# Autodesk Inventor assembly: Gearbox #2
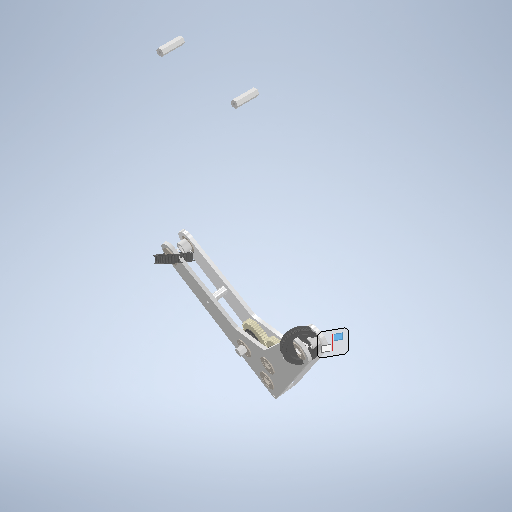
[picture p0: Inventor's stored thumbnail of the model, 512x512]
Saved by Autodesk Inventor 2025.1 (Build 291241020, 241B)
## iProperties
Created: 2024-09-29
Part Number: Gearbox #2
Document SubType Name: Assembly
Designer: xmand
Author: xmand
## Documents named in this file (13)
- C:\Users\xmand\OneDrive\Documents\GitHub\1622-2024-Assignments\Xavier Daza\Gearbox #2.iam
- C:\Users\xmand\OneDrive\Documents\GitHub\1622-2024-Assignments\Xavier Daza\Gearbox #1\Gearbox #2 Top Plate.ipt
- C:\Users\xmand\OneDrive\Documents\GitHub\1622-2024-Assignments\Xavier Daza\Gearbox #1\Gearbox #2 Plate.ipt
- C:\Users\xmand\OneDrive\Documents\GitHub\1622-2024-Assignments\Xavier Daza\Gearbox #1\WCP-0188 (1).ipt
- C:\Users\xmand\Downloads\WCP-0709\WCP-0709\WCP-0709.ipt
- C:\Users\xmand\Downloads\WCP-0783\WCP-0783\WCP-0783.ipt
- C:\Users\xmand\Downloads\WCP-0564\WCP-0564\WCP-0564.ipt
- C:\Users\xmand\Downloads\WCP-0990\WCP-0990\WCP-0990.ipt
- C:\Users\xmand\OneDrive\Documents\GitHub\1622-2024-Assignments\Xavier Daza\WCP-0787-01.ipt
- C:\Users\xmand\OneDrive\Documents\GitHub\1622-2024-Assignments\Xavier Daza\10-32 0.5 1.131 Inch Stand Off.ipt
- C:\Users\xmand\OneDrive\Documents\GitHub\1622-2024-Assignments\Xavier Daza\0.498 Spacer 0.5 Hex.ipt
- C:\Users\xmand\OneDrive\Documents\GitHub\1622-2024-Assignments\Xavier Daza\0.633 Spacer 0.5 Hex.ipt
- C:\Users\xmand\OneDrive\Documents\GitHub\1622-2024-Assignments\Xavier Daza\Hex shaft 0.201 and 0.500.ipt
## Components (32 placed, 12 different names)
1. Gearbox #2 Top Plate:1 — Mate:1, Mate:2, Insert:6, Insert:7, Insert:8, Insert:9, Insert:10, Mate:17, Mate:18, Mate:19
2. Gearbox #2 Plate:1 — Mate:1, Mate:2, Insert:1, Insert:2, Insert:3, Insert:4, Insert:5, Mate:15, Mate:16
3. WCP-0188 (1):1 — Mate:5, Angle:2, Angle:4, Mate:7, Angle:8
4. WCP-0188 (1):2 — Mate:3, Angle:1, Angle:5, Mate:6, Angle:10
5. WCP-0709:1 — Mate:4, Angle:3, Angle:6
6. WCP-0783:1 — Insert:7, Angle:4, Mate:10
7. WCP-0783:2 — Insert:4, Mate:4, Angle:3
8. WCP-0783:3 — Insert:3, Mate:3, Angle:1
9. WCP-0783:4 — Insert:2, Angle:9, Mate:20
10. WCP-0783:5 — Insert:1, Mate:5, Angle:2, Angle:11, Insert:11
11. WCP-0783:6 — Insert:6, Mate:11
12. WCP-0783:7 — Insert:8, Angle:6, Mate:22
13. WCP-0783:8 — Insert:10, Mate:8
14. WCP-0783:9 — Insert:9, Angle:5, Mate:9
15. WCP-0783:10 — Insert:5, Mate:21
16. WCP-0564:1 — Mate:7, Angle:8, Mate:12
17. WCP-0564:2 — Mate:6, Angle:10
18. WCP-0990:1 — Angle:9, Mate:14
19. WCP-0990:2 — Mate:13
20. WCP-0787-01:1 — Mate:10, Mate:12
21. WCP-0787-01:2 — Mate:11, Mate:14
22. WCP-0787-01:3 — Mate:9
23. WCP-0787-01:4 — Mate:8, Mate:13
24. 10-32 0.5 1.131 Inch Stand Off:1 — Mate:19
25. 10-32 0.5 1.131 Inch Stand Off:2 — Mate:15, Mate:18
26. 10-32 0.5 1.131 Inch Stand Off:3 — Mate:16, Mate:17
27. 0.498 Spacer 0.5 Hex:1 — Mate:20
28. 0.498 Spacer 0.5 Hex:2 — Mate:21
29. 0.633 Spacer 0.5 Hex:1 — Mate:22
30. Hex shaft 0.201 and 0.500:1
31. Hex shaft 0.201 and 0.500:2
32. Hex shaft 0.201 and 0.500:3 — Angle:11, Insert:11
## Relationships (43: Mate 22, Insert 11, Angle 10)
- Mate:1: Gearbox #2 Top Plate:1 ↔ Gearbox #2 Plate:1
- Mate:2: Gearbox #2 Top Plate:1 ↔ Gearbox #2 Plate:1
- Insert:1: Gearbox #2 Plate:1 ↔ WCP-0783:5
- Insert:2: Gearbox #2 Plate:1 ↔ WCP-0783:4
- Insert:3: Gearbox #2 Plate:1 ↔ WCP-0783:3
- Insert:4: Gearbox #2 Plate:1 ↔ WCP-0783:2
- Insert:5: Gearbox #2 Plate:1 ↔ WCP-0783:10
- Insert:6: Gearbox #2 Top Plate:1 ↔ WCP-0783:6
- Insert:7: Gearbox #2 Top Plate:1 ↔ WCP-0783:1
- Insert:8: Gearbox #2 Top Plate:1 ↔ WCP-0783:7
- Insert:9: Gearbox #2 Top Plate:1 ↔ WCP-0783:9
- Insert:10: Gearbox #2 Top Plate:1 ↔ WCP-0783:8
- Mate:3: WCP-0188 (1):2 ↔ WCP-0783:3
- Mate:4: WCP-0709:1 ↔ WCP-0783:2
- Mate:5: WCP-0188 (1):1 ↔ WCP-0783:5
- Angle:1 (0 deg): WCP-0188 (1):2 ↔ WCP-0783:3
- Angle:2 (0 deg): WCP-0188 (1):1 ↔ WCP-0783:5
- Angle:3 (0 deg): WCP-0709:1 ↔ WCP-0783:2
- Angle:4 (0 deg): WCP-0188 (1):1 ↔ WCP-0783:1
- Angle:5 (0 deg): WCP-0188 (1):2 ↔ WCP-0783:9
- Angle:6 (0 deg): WCP-0709:1 ↔ WCP-0783:7
- Mate:6: WCP-0188 (1):2 ↔ WCP-0564:2
- Mate:7: WCP-0188 (1):1 ↔ WCP-0564:1
- Angle:8 (0 deg): WCP-0188 (1):1 ↔ WCP-0564:1
- Angle:9 (0 deg): WCP-0783:4 ↔ WCP-0990:1
- Angle:10 (0 deg): WCP-0188 (1):2 ↔ WCP-0564:2
- Mate:8: WCP-0783:8 ↔ WCP-0787-01:4
- Mate:9: WCP-0783:9 ↔ WCP-0787-01:3
- Mate:10: WCP-0783:1 ↔ WCP-0787-01:1
- Mate:11: WCP-0783:6 ↔ WCP-0787-01:2
- Mate:12: WCP-0564:1 ↔ WCP-0787-01:1
- Mate:13: WCP-0990:2 ↔ WCP-0787-01:4
- Mate:14: WCP-0990:1 ↔ WCP-0787-01:2
- Mate:15: Gearbox #2 Plate:1 ↔ 10-32 0.5 1.131 Inch Stand Off:2
- Mate:16: Gearbox #2 Plate:1 ↔ 10-32 0.5 1.131 Inch Stand Off:3
- Mate:17: Gearbox #2 Top Plate:1 ↔ 10-32 0.5 1.131 Inch Stand Off:3
- Mate:18: Gearbox #2 Top Plate:1 ↔ 10-32 0.5 1.131 Inch Stand Off:2
- Mate:19: Gearbox #2 Top Plate:1 ↔ 10-32 0.5 1.131 Inch Stand Off:1
- Mate:20: WCP-0783:4 ↔ 0.498 Spacer 0.5 Hex:1
- Mate:21: WCP-0783:10 ↔ 0.498 Spacer 0.5 Hex:2
- Mate:22: WCP-0783:7 ↔ 0.633 Spacer 0.5 Hex:1
- Angle:11 (0 deg): WCP-0783:5 ↔ Hex shaft 0.201 and 0.500:3
- Insert:11: WCP-0783:5 ↔ Hex shaft 0.201 and 0.500:3
